# Autodesk Inventor assembly: Rover Swerve Drive Mount 1.19
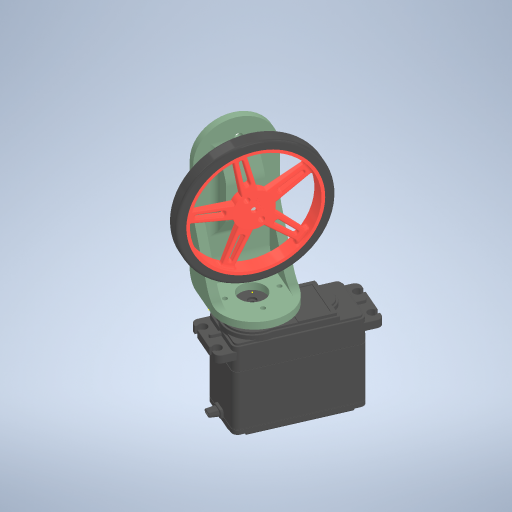
[picture p0: Inventor's stored thumbnail of the model, 512x512]
Saved by Autodesk Inventor 2024 (Build 280153000, 153)
## iProperties
Created: 2024-01-13
Part Number: Rover Swerve Drive Mount 1.19
Document SubType Name: Assembly
Designer: student
Author: student
## Documents named in this file (7)
- F:\Rover, TRACER\Rover Swerve Drive\Rover Swerve Drive Mount 1.19.iam
- F:\Rover, TRACER\Rover Swerve Drive\Servo 775 (with Spline).iam
- F:\Rover, TRACER\Rover Swerve Drive\dcmotorLBracklet.ipt
- F:\Rover, TRACER\Rover Swerve Drive\N20Motor.iam
- F:\Rover, TRACER\Rover Swerve Drive\RedWheel.ipt
- F:\Rover, TRACER\Rover Swerve Drive\N20Bracklet- Left.ipt
- F:\Rover, TRACER\Rover Swerve Drive\N20Bracklet-Holder.ipt
## Components (6 placed, 6 different names)
1. Servo 775 (with Spline):1 [sub-assembly] — Flush:1, Mate:2, Angle:1
2. dcmotorLBracklet:1 — Flush:1, Mate:2, Angle:1, Mate:7, Mate:8, Mate:9, Mate:12, Angle:2
3. N20Motor:1 [sub-assembly] — Mate:7, Mate:8, Mate:10, Mate:11, Flush:3
4. RedWheel:1 — Mate:9, Mate:10
5. N20Bracklet- Left:1 — Mate:11, Mate:12, Flush:3, Flush:4, Angle:2, Mate:13, Mate:14
6. N20Bracklet-Holder:1 — Flush:4, Mate:13, Mate:14
## Relationships (14: Mate 9, Flush 3, Angle 2)
- Flush:1: Servo 775 (with Spline):1 ↔ dcmotorLBracklet:1
- Mate:2: Servo 775 (with Spline):1 ↔ dcmotorLBracklet:1
- Angle:1 (0 deg): Servo 775 (with Spline):1 ↔ dcmotorLBracklet:1
- Mate:7: dcmotorLBracklet:1 ↔ N20Motor:1
- Mate:8: dcmotorLBracklet:1 ↔ N20Motor:1
- Mate:9: dcmotorLBracklet:1 ↔ RedWheel:1
- Mate:10: N20Motor:1 ↔ RedWheel:1
- Mate:11: N20Motor:1 ↔ N20Bracklet- Left:1
- Mate:12: dcmotorLBracklet:1 ↔ N20Bracklet- Left:1
- Flush:3: N20Motor:1 ↔ N20Bracklet- Left:1
- Flush:4: N20Bracklet- Left:1 ↔ N20Bracklet-Holder:1
- Angle:2 (0 deg): dcmotorLBracklet:1 ↔ N20Bracklet- Left:1
- Mate:13: N20Bracklet- Left:1 ↔ N20Bracklet-Holder:1
- Mate:14: N20Bracklet- Left:1 ↔ N20Bracklet-Holder:1
